# Autodesk Inventor assembly: BLDC motor
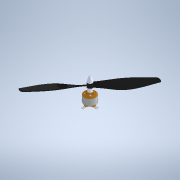
[picture p0: Inventor's stored thumbnail of the model, 180x180]
Saved by Autodesk Inventor 2021 (Build 250183000, 183)
## iProperties
Created: 2019-08-02
Part Number: BLDC motor
Document SubType Name: Assembly
Designer: leejun
Sending System: SolidWorks 2018
Last Author: User
Last Saved: 2019-08-02
Author: leejun
## Documents named in this file (7)
- C:\Users\leejun\Desktop\bldc-motor-and-propeller-1.snapshot.1\BLDC motor\BLDC motor.iam
- C:\Users\leejun\Desktop\bldc-motor-and-propeller-1.snapshot.1\BLDC motor\motor_stator.iam
- C:\Users\leejun\Desktop\bldc-motor-and-propeller-1.snapshot.1\BLDC motor\motor_rotor.iam
- C:\Users\leejun\Desktop\bldc-motor-and-propeller-1.snapshot.1\BLDC motor\clamp.ipt
- C:\Users\leejun\Desktop\bldc-motor-and-propeller-1.snapshot.1\BLDC motor\propeller.ipt
- C:\Users\leejun\Desktop\bldc-motor-and-propeller-1.snapshot.1\BLDC motor\prop adapter.ipt
- C:\Users\leejun\Desktop\bldc-motor-and-propeller-1.snapshot.1\BLDC motor\adapter nut.ipt
## Components (6 placed, 6 different names)
1. motor_stator:1 [sub-assembly] — 메이트:7, 메이트:8, 메이트:9, 메이트:10, 메이트:11
2. motor_rotor:1 [sub-assembly] — 메이트:1, 메이트:4, 메이트:7, 메이트:8, 회전:1
3. clamp:1 — 메이트:9, 메이트:10, 메이트:11
4. propeller:1 — 메이트:2, 메이트:5, 메이트:6, 회전:2
5. adapter nut:1 — 메이트:3, 메이트:6, 회전:3
6. prop adapter:1 — 메이트:1, 메이트:2, 메이트:3, 메이트:4, 메이트:5, 회전:1, 회전:2, 회전:3
## Relationships (14: Mate 11, RelateRotation 3)
- 메이트:1 [Mate]: motor_rotor:1 ↔ prop adapter:1
- 메이트:2 [Mate]: propeller:1 ↔ prop adapter:1
- 메이트:3 [Mate]: adapter nut:1 ↔ prop adapter:1
- 메이트:4 [Mate] (1 mm): motor_rotor:1 ↔ prop adapter:1
- 메이트:5 [Mate] (1 mm): propeller:1 ↔ prop adapter:1
- 메이트:6 [Mate] (0.5 mm): propeller:1 ↔ adapter nut:1
- 메이트:7 [Mate]: motor_stator:1 ↔ motor_rotor:1
- 메이트:8 [Mate] (0.1 mm): motor_stator:1 ↔ motor_rotor:1
- 메이트:9 [Mate]: motor_stator:1 ↔ clamp:1
- 메이트:10 [Mate]: motor_stator:1 ↔ clamp:1
- 메이트:11 [Mate]: motor_stator:1 ↔ clamp:1
- 회전:1 [RelateRotation] (1 ul): motor_rotor:1 ↔ prop adapter:1
- 회전:2 [RelateRotation] (1 ul): propeller:1 ↔ prop adapter:1
- 회전:3 [RelateRotation] (1 ul): adapter nut:1 ↔ prop adapter:1
